# Autodesk Inventor assembly: Conector
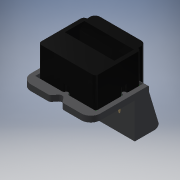
[picture p0: Inventor's stored thumbnail of the model, 180x180]
Saved by Autodesk Inventor 2018 (Build 220112000, 112)
## iProperties
Created: 2020-08-08
Part Number: Conector
Document SubType Name: Assembly
Designer: sawer
Author: sawer
## iProperties of the stored document PinSocket_1x06_P2.54mm_Vertical.ipt
Company: FreeCAD
Created: 2017-11-27
Part Number: PinSocket_1x06_P2.54mm_Vertical
Material: Generic
Description: model of PinSocket_1x06_P2.54mm_Vertical
Document SubType Name: Modeling
Designer: sawer
Density: 1 g/cm^3
Appearance: Default
Sending System: kicad StepUp
Preprocessor: OCC
Title: PinSocket_1x06_P2.54mm_Vertical.step
Author: Terje Io
## Documents named in this file (6)
- **C:\Documentos\3D\Sensor de Flujo\Conector.iam*LocalDocs*xAfzfdlh0MmzrugkxNvt1n0tmSc*PinSocket_1x06_P2.54mm_Vertical.ipt
- C:\Documentos\3D\Sensor de Flujo\Conector.iam
- C:\Documentos\3D\Sensor de Flujo\TUBE_PCB.ipt
- C:\Documentos\3D\Sensor de Flujo\PCB_SMF3300.ipt
- C:\Documentos\3D\Sensor de Flujo\SMF3300_CONECTOR.ipt
- C:\Program Files\KiCad\share\kicad\modules\packages3d\Connector_PinSocket_2.54mm.3dshapes\PinSocket_1x06_P2.54mm_Vertical.step
## Components (4 placed, 4 different names)
1. TUBE_PCB:1 — Mate:1
2. PCB_SMF3300:1 — Mate:1, Mate:2
3. SMF3300_CONECTOR:1 — Mate:2
4. PinSocket_1x06_P2.54mm_Vertical:1
## Relationships (2: Mate 2)
- Mate:1 (0.5 mm): TUBE_PCB:1 ↔ PCB_SMF3300:1
- Mate:2: PCB_SMF3300:1 ↔ SMF3300_CONECTOR:1
